# Autodesk Inventor assembly: assy_parkinglot_front_right
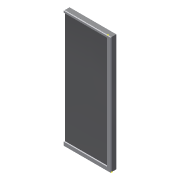
[picture p0: Inventor's stored thumbnail of the model, 180x180]
Saved by Autodesk Inventor 2018 (Build 220112000, 112)
## iProperties
Created: 2017-11-13
Part Number: assy_parkinglot_front_right
Document SubType Name: Assembly
Designer: Platform
Author: Platform
## Documents named in this file (5)
- C:\Users\Platform\Desktop\autorace_track\track_model\autorace_rbizchallenge2017\assembled\assy_parkinglot_front_right.iam
- C:\Users\Platform\Desktop\autorace_track\track_model\autorace_rbizchallenge2017\parts\ipt\upper_plate_parking2 v1.ipt
- C:\Users\Platform\Desktop\autorace_track\track_model\autorace_rbizchallenge2017\parts\ipt\straight_line.ipt
- C:\Users\Platform\Desktop\autorace_track\track_model\autorace_rbizchallenge2017\parts\ipt\line_edge_parkinglot_2_1.ipt
- C:\Users\Platform\Desktop\autorace_track\track_model\autorace_rbizchallenge2017\parts\ipt\line_edge_parkinglot_2_2.ipt
## Components (4 placed, 4 different names)
1. upper_plate_parking2 v1:1 — Mate:1, Flush:1, Flush:2, Mate:2, Flush:3, Flush:4, Mate:5
2. straight_line:1 — Mate:1, Flush:1, Flush:2, Mate:3, Mate:4
3. line_edge_parkinglot_2_1:1 — Mate:2, Flush:3, Mate:3
4. line_edge_parkinglot_2_2:1 — Mate:4, Flush:4, Mate:5
## Relationships (9: Mate 5, Flush 4)
- Mate:1: upper_plate_parking2 v1:1 ↔ straight_line:1
- Flush:1: upper_plate_parking2 v1:1 ↔ straight_line:1
- Flush:2: upper_plate_parking2 v1:1 ↔ straight_line:1
- Mate:2: upper_plate_parking2 v1:1 ↔ line_edge_parkinglot_2_1:1
- Flush:3: upper_plate_parking2 v1:1 ↔ line_edge_parkinglot_2_1:1
- Mate:3: straight_line:1 ↔ line_edge_parkinglot_2_1:1
- Mate:4: straight_line:1 ↔ line_edge_parkinglot_2_2:1
- Flush:4: upper_plate_parking2 v1:1 ↔ line_edge_parkinglot_2_2:1
- Mate:5: upper_plate_parking2 v1:1 ↔ line_edge_parkinglot_2_2:1
